# Autodesk Inventor assembly: HCMUTE-CDT23-PLXR_KXL
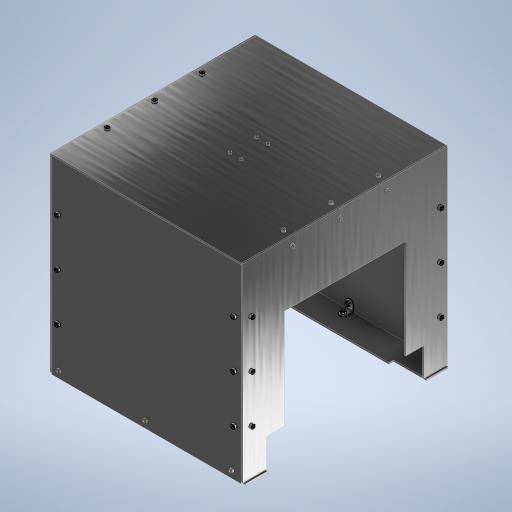
[picture p0: Inventor's stored thumbnail of the model, 512x512]
Saved by Autodesk Inventor 2023 (Build 270158000, 158)
## iProperties
Created: 2023-11-19
Part Number: HCMUTE-CDT23-PLXR_KXL
Document SubType Name: Assembly
Designer: havie
Mass: 52555 g
Surface Area: 83477.5 cm^2
Volume: 13075.1 cm^3
Density: 4.01946 g/cm^3
Author: havie
## Documents named in this file (15)
- D:\DO_AN_CDT\1.1. PART\HCMUTE-CDT23-PLXR_KXL.iam
- C:\Users\havie\Documents\Inventor\Content Center Files\R2023\en-US\ISO 4762(2)\ISO 4762 - M6 x 10ISO.ipt
- C:\Users\havie\Documents\Inventor\Content Center Files\R2023\en-US\ISO 4762(2)\ISO 4762 - M5 x 12ISO.ipt
- D:\DO_AN_CDT\1.1. PART\CAMERA\Assembly_HCMUTE-CDT23-CAMERA_C270Logitech c270 Assembly.iam
- D:\DO_AN_CDT\1.1. PART\HCMUTE-CDT23-KXL_A01.ipt
- C:\Users\havie\Documents\Inventor\Content Center Files\R2023\en-US\ISO 4032(2)\ISO 4032 - M5 - ISO.ipt
- D:\DO_AN_CDT\1.1. PART\2309HCMUTE-CDT23-KXL_GA-VUONG.ipt
- D:\DO_AN_CDT\1.1. PART\HCMUTE-CDT23-KXL_A02.ipt
- D:\DO_AN_CDT\1.1. PART\HCMUTE-CDT23-KXL_A03.ipt
- D:\DO_AN_CDT\1.1. PART\HCMUTE-CDT23-KXL_A04.ipt
- D:\DO_AN_CDT\1.1. PART\HCMUTE-CDT23-KXL_A05.ipt
- D:\DO_AN_CDT\1.1. PART\CBIEN\Assembly_HCMUTE-CDT23-CB_E3F-DS30C4.iam
- D:\DO_AN_CDT\1.1. PART\HCMUTE-CDT23-KXL_A06.ipt
- C:\Users\havie\Documents\Inventor\Content Center Files\R2023\en-US\ISO 4762(2)\ISO 4762 - M4 x 16ISO.ipt
- C:\Users\havie\Documents\Inventor\Content Center Files\R2023\en-US\ISO 4032(2)\ISO 4032 - M4 - ISO.ipt
## Components (144 placed, 14 different names)
1. HCMUTE-CDT23-KXL_A01:1 — Mate:288, Flush:55, Mate:289, Mate:290, Mate:291, Mate:292, Mate:293, Flush:57, Mate:313, Mate:360
2. 2309HCMUTE-CDT23-KXL_GA-VUONG:1 — Mate:288, Flush:55, Mate:289, Flush:56, Mate:476, Mate:477
3. 2309HCMUTE-CDT23-KXL_GA-VUONG:2 — Mate:290, Flush:56, Mate:291
4. 2309HCMUTE-CDT23-KXL_GA-VUONG:3 — Mate:292, Mate:293, Flush:57, Mate:478
5. ISO 4032 M5:1
6. HCMUTE-CDT23-KXL_A03:1 — Mate:313, Mate:316, Mate:319, Flush:61, Flush:62, Mate:338, Mate:355, Mate:356, Mate:370, Symmetry:3
7. HCMUTE-CDT23-KXL_A02:2 — Mate:319, Flush:61, Flush:62, Mate:333, Mate:334, Mate:335, Flush:69, Mate:336, Mate:337, Mate:341, Mate:342, Mate:347, Mate:348, Mate:351, Mate:352, Mate:474, Mate:475
8. HCMUTE-CDT23-KXL_A01:2 — Mate:331
9. HCMUTE-CDT23-KXL_A04:1 — Mate:360, Mate:361, Mate:362, Mate:363, Mate:364, Mate:373, Mate:380, Mate:381, Symmetry:3
10. HCMUTE-CDT23-KXL_A05:1 — Mate:370, Mate:371, Flush:72, Mate:372, Mate:374, Mate:375, Mate:382, Mate:383, Mate:384, Mate:385, Mate:386, Mate:481, Mate:482, Mate:483, Mate:484, Mate:485, Mate:486, Mate:487, Mate:488
11. ISO 4762 M5 x 12:44
12. ISO 4032 M5:40
13. ISO 4032 M5:41
14. ISO 4762 M5 x 12:45
15. ISO 4762 M5 x 12:46
16. ISO 4032 M5:42
17. ISO 4032 M5:43
18. ISO 4762 M5 x 12:47
19. ISO 4762 M5 x 12:48
20. ISO 4032 M5:44
21. ISO 4032 M5:45
22. ISO 4762 M5 x 12:49
23. Assembly_HCMUTE-CDT23-CAMERA_C270Logitech c270 Assembly:2 [sub-assembly] — Mate:384, Mate:385, Mate:386, Mate:493, Mate:494, Mate:495, Mate:496
24. Assembly_HCMUTE-CDT23-CB_E3F-DS30C4:2 [sub-assembly] — Mate:474, Mate:475
25. HCMUTE-CDT23-KXL_A06:1 — Mate:476, Mate:477, Mate:478
26. ISO 4032 M5:60 — Mate:479
27. ISO 4032 M5:61 — Mate:480
28. ISO 4762 M5 x 12:76 — Mate:480
29. ISO 4762 M5 x 12:77 — Mate:479
30. ISO 4032 M5:62
31. ISO 4032 M5:63
32. ISO 4762 M5 x 12:78
33. ISO 4762 M5 x 12:79
34. ISO 4032 M5:64
35. ISO 4032 M5:65
36. ISO 4762 M5 x 12:80
37. ISO 4762 M5 x 12:81
38. ISO 4762 M4 x 16:1 — Mate:483, Mate:486, Mate:490
39. ISO 4762 M4 x 16:2 — Mate:482, Mate:487, Mate:489
40. ISO 4762 M4 x 16:3 — Mate:481, Mate:488, Mate:491
41. ISO 4762 M4 x 16:4 — Mate:484, Mate:485, Mate:492
42. ISO 4032 M4:1 — Mate:489, Mate:494
43. ISO 4032 M4:2 — Mate:490, Mate:496
44. ISO 4032 M4:3 — Mate:491, Mate:493
45. ISO 4032 M4:4 — Mate:492, Mate:495
46. ISO 4032 M5:10 — Mate:317, Mate:318
47. ISO 4762 M5 x 12:14 — Mate:315, Mate:316, Mate:318
48. ISO 4032 M5:11
49. ISO 4762 M5 x 12:15
50. ISO 4032 M5:12
51. ISO 4762 M5 x 12:16
52. ISO 4762 M6 x 10:16
53. ISO 4762 M6 x 10:15
54. ISO 4762 M6 x 10:17
55. ISO 4762 M6 x 10:18
56. ISO 4762 M6 x 10:19
57. ISO 4762 M6 x 10:20
58. 2309HCMUTE-CDT23-KXL_GA-VUONG:10 — Mate:331, Mate:333, Mate:339, Mate:343, Mate:345
59. 2309HCMUTE-CDT23-KXL_GA-VUONG:13
60. 2309HCMUTE-CDT23-KXL_GA-VUONG:14
61. 2309HCMUTE-CDT23-KXL_GA-VUONG:11 — Mate:334, Mate:335, Flush:69, Mate:349
62. 2309HCMUTE-CDT23-KXL_GA-VUONG:12 — Mate:336, Mate:337, Mate:338, Mate:354, Mate:357
63. 2309HCMUTE-CDT23-KXL_GA-VUONG:15
64. 2309HCMUTE-CDT23-KXL_GA-VUONG:16
65. 2309HCMUTE-CDT23-KXL_GA-VUONG:17 — Mate:367
66. 2309HCMUTE-CDT23-KXL_GA-VUONG:18
67. ISO 4032 M5:15 — Mate:343, Mate:344
68. ISO 4032 M5:16 — Mate:345, Mate:346
69. ISO 4762 M5 x 12:20 — Mate:341, Mate:342, Mate:346
70. ISO 4762 M5 x 12:17 — Mate:339, Mate:344
71. ISO 4032 M5:17
72. ISO 4032 M5:18
73. ISO 4762 M5 x 12:21
74. ISO 4762 M5 x 12:22
75. ISO 4032 M5:19
76. ISO 4032 M5:20
77. ISO 4762 M5 x 12:23
78. ISO 4762 M5 x 12:24
79. ISO 4762 M5 x 12:18 — Mate:347, Mate:348, Mate:350
80. ISO 4032 M5:14 — Mate:349, Mate:350
81. ISO 4762 M5 x 12:25
82. ISO 4032 M5:21
83. ISO 4762 M5 x 12:26
84. ISO 4032 M5:22
85. ISO 4032 M5:13 — Mate:353, Mate:354
86. ISO 4762 M5 x 12:19 — Mate:351, Mate:352, Mate:353
87. ISO 4762 M5 x 12:27 — Mate:355, Mate:356, Mate:358
88. ISO 4032 M5:23 — Mate:357, Mate:358
89. ISO 4032 M5:24
90. ISO 4762 M5 x 12:28
91. ISO 4762 M5 x 12:29
92. ISO 4032 M5:25
93. ISO 4032 M5:26
94. ISO 4762 M5 x 12:30
95. ISO 4762 M5 x 12:31
96. ISO 4032 M5:27
97. ISO 4032 M5:29 — Mate:367, Mate:368
98. ISO 4762 M5 x 12:32 — Mate:361, Mate:362, Mate:368
99. ISO 4032 M5:28 — Mate:365, Mate:366
100. ISO 4762 M5 x 12:33 — Mate:363, Mate:364, Mate:366
101. ISO 4032 M5:30
102. ISO 4762 M5 x 12:34
103. ISO 4032 M5:31
104. ISO 4762 M5 x 12:35
105. ISO 4032 M5:32
106. ISO 4762 M5 x 12:36
107. ISO 4032 M5:33
108. ISO 4762 M5 x 12:37
109. 2309HCMUTE-CDT23-KXL_GA-VUONG:19 — Mate:371, Flush:72, Mate:372
110. 2309HCMUTE-CDT23-KXL_GA-VUONG:20
111. 2309HCMUTE-CDT23-KXL_GA-VUONG:21
112. 2309HCMUTE-CDT23-KXL_GA-VUONG:22 — Mate:373, Mate:374, Mate:375, Mate:376, Mate:377, Mate:378, Mate:379
113. 2309HCMUTE-CDT23-KXL_GA-VUONG:23
114. 2309HCMUTE-CDT23-KXL_GA-VUONG:24
115. ISO 4762 M5 x 12:38 — Mate:380, Mate:381
116. ISO 4032 M5:34 — Mate:376, Mate:377
117. ISO 4032 M5:35 — Mate:378, Mate:379
118. ISO 4762 M5 x 12:39 — Mate:382, Mate:383
119. ISO 4762 M5 x 12:40
120. ISO 4032 M5:36
121. ISO 4032 M5:37
122. ISO 4762 M5 x 12:41
123. ISO 4762 M5 x 12:42
124. ISO 4032 M5:38
125. ISO 4032 M5:39
126. ISO 4762 M5 x 12:43
127. 2309HCMUTE-CDT23-KXL_GA-VUONG:4 — Mate:309, Mate:365
128. ISO 4032 M5:5 — Mate:309, Mate:310
129. ISO 4762 M5 x 12:8 — Mate:310
130. 2309HCMUTE-CDT23-KXL_GA-VUONG:30
131. ISO 4032 M5:56
132. ISO 4762 M5 x 12:72
133. 2309HCMUTE-CDT23-KXL_GA-VUONG:31
134. ISO 4032 M5:57
135. ISO 4762 M5 x 12:73
136. ISO 4032 M5:4 — Mate:311, Mate:312
137. 2309HCMUTE-CDT23-KXL_GA-VUONG:7 — Mate:312, Mate:315, Mate:317
138. ISO 4762 M5 x 12:9 — Mate:311
139. ISO 4032 M5:58
140. 2309HCMUTE-CDT23-KXL_GA-VUONG:32
141. ISO 4762 M5 x 12:74
142. ISO 4032 M5:59
143. 2309HCMUTE-CDT23-KXL_GA-VUONG:33
144. ISO 4762 M5 x 12:75
## Component patterns: (3 elements, first: ISO 4032 M5:10 + ISO 4762 M5 x 12:14), (3 elements, first: ISO 4762 M6 x 10:16 + ISO 4762 M6 x 10:15), (3 elements, first: 2309HCMUTE-CDT23-KXL_GA-VUONG:10), (3 elements, first: 2309HCMUTE-CDT23-KXL_GA-VUONG:11 + 2309HCMUTE-CDT23-KXL_GA-VUONG:12), (3 elements, first: ISO 4032 M5:15 + ISO 4032 M5:16 + ISO 4762 M5 x 12:20 + ISO 4762 M5 x 12:17), (3 elements, first: ISO 4762 M5 x 12:18 + ISO 4032 M5:14), (3 elements, first: ISO 4032 M5:13 + ISO 4762 M5 x 12:19 + ISO 4762 M5 x 12:27 + ISO 4032 M5:23), (3 elements, first: ISO 4032 M5:29 + ISO 4762 M5 x 12:32 + ISO 4032 M5:28 + ISO 4762 M5 x 12:33), (3 elements, first: 2309HCMUTE-CDT23-KXL_GA-VUONG:19), (3 elements, first: 2309HCMUTE-CDT23-KXL_GA-VUONG:22), (3 elements, first: ISO 4762 M5 x 12:38 + ISO 4032 M5:34 + ISO 4032 M5:35 + ISO 4762 M5 x 12:39), (3 elements, first: 2309HCMUTE-CDT23-KXL_GA-VUONG:4 + ISO 4032 M5:5 + ISO 4762 M5 x 12:8), (3 elements, first: ISO 4032 M5:4 + 2309HCMUTE-CDT23-KXL_GA-VUONG:7 + ISO 4762 M5 x 12:9)
## Relationships (99: Mate 91, Flush 7, Symmetry 1)
- Mate:288: HCMUTE-CDT23-KXL_A01:1 ↔ 2309HCMUTE-CDT23-KXL_GA-VUONG:1
- Flush:55: HCMUTE-CDT23-KXL_A01:1 ↔ 2309HCMUTE-CDT23-KXL_GA-VUONG:1
- Mate:289: HCMUTE-CDT23-KXL_A01:1 ↔ 2309HCMUTE-CDT23-KXL_GA-VUONG:1
- Mate:290: HCMUTE-CDT23-KXL_A01:1 ↔ 2309HCMUTE-CDT23-KXL_GA-VUONG:2
- Flush:56: 2309HCMUTE-CDT23-KXL_GA-VUONG:1 ↔ 2309HCMUTE-CDT23-KXL_GA-VUONG:2
- Mate:291: HCMUTE-CDT23-KXL_A01:1 ↔ 2309HCMUTE-CDT23-KXL_GA-VUONG:2
- Mate:292: HCMUTE-CDT23-KXL_A01:1 ↔ 2309HCMUTE-CDT23-KXL_GA-VUONG:3
- Mate:293: HCMUTE-CDT23-KXL_A01:1 ↔ 2309HCMUTE-CDT23-KXL_GA-VUONG:3
- Flush:57: HCMUTE-CDT23-KXL_A01:1 ↔ 2309HCMUTE-CDT23-KXL_GA-VUONG:3
- Mate:309: 2309HCMUTE-CDT23-KXL_GA-VUONG:4 ↔ ISO 4032 M5:5
- Mate:310: ISO 4032 M5:5 ↔ ISO 4762 M5 x 12:8
- Mate:311: ISO 4032 M5:4 ↔ ISO 4762 M5 x 12:9
- Mate:312: ISO 4032 M5:4 ↔ 2309HCMUTE-CDT23-KXL_GA-VUONG:7
- Mate:313: HCMUTE-CDT23-KXL_A01:1 ↔ HCMUTE-CDT23-KXL_A03:1
- Mate:315: ISO 4762 M5 x 12:14 ↔ 2309HCMUTE-CDT23-KXL_GA-VUONG:7
- Mate:316: HCMUTE-CDT23-KXL_A03:1 ↔ ISO 4762 M5 x 12:14
- Mate:317: ISO 4032 M5:10 ↔ 2309HCMUTE-CDT23-KXL_GA-VUONG:7
- Mate:318: ISO 4032 M5:10 ↔ ISO 4762 M5 x 12:14
- Mate:319: HCMUTE-CDT23-KXL_A03:1 ↔ HCMUTE-CDT23-KXL_A02:2
- Flush:61: HCMUTE-CDT23-KXL_A03:1 ↔ HCMUTE-CDT23-KXL_A02:2
- Flush:62 (3 mm): HCMUTE-CDT23-KXL_A03:1 ↔ HCMUTE-CDT23-KXL_A02:2
- Mate:331: HCMUTE-CDT23-KXL_A01:2 ↔ 2309HCMUTE-CDT23-KXL_GA-VUONG:10
- Mate:333: HCMUTE-CDT23-KXL_A02:2 ↔ 2309HCMUTE-CDT23-KXL_GA-VUONG:10
- Mate:334: HCMUTE-CDT23-KXL_A02:2 ↔ 2309HCMUTE-CDT23-KXL_GA-VUONG:11
- Mate:335: HCMUTE-CDT23-KXL_A02:2 ↔ 2309HCMUTE-CDT23-KXL_GA-VUONG:11
- Flush:69: HCMUTE-CDT23-KXL_A02:2 ↔ 2309HCMUTE-CDT23-KXL_GA-VUONG:11
- Mate:336: HCMUTE-CDT23-KXL_A02:2 ↔ 2309HCMUTE-CDT23-KXL_GA-VUONG:12
- Mate:337: HCMUTE-CDT23-KXL_A02:2 ↔ 2309HCMUTE-CDT23-KXL_GA-VUONG:12
- Mate:338: HCMUTE-CDT23-KXL_A03:1 ↔ 2309HCMUTE-CDT23-KXL_GA-VUONG:12
- Mate:339: 2309HCMUTE-CDT23-KXL_GA-VUONG:10 ↔ ISO 4762 M5 x 12:17
- Mate:341: HCMUTE-CDT23-KXL_A02:2 ↔ ISO 4762 M5 x 12:20
- Mate:342: HCMUTE-CDT23-KXL_A02:2 ↔ ISO 4762 M5 x 12:20
- Mate:343: 2309HCMUTE-CDT23-KXL_GA-VUONG:10 ↔ ISO 4032 M5:15
- Mate:344: ISO 4032 M5:15 ↔ ISO 4762 M5 x 12:17
- Mate:345: 2309HCMUTE-CDT23-KXL_GA-VUONG:10 ↔ ISO 4032 M5:16
- Mate:346: ISO 4032 M5:16 ↔ ISO 4762 M5 x 12:20
- Mate:347: HCMUTE-CDT23-KXL_A02:2 ↔ ISO 4762 M5 x 12:18
- Mate:348: HCMUTE-CDT23-KXL_A02:2 ↔ ISO 4762 M5 x 12:18
- Mate:349: 2309HCMUTE-CDT23-KXL_GA-VUONG:11 ↔ ISO 4032 M5:14
- Mate:350: ISO 4762 M5 x 12:18 ↔ ISO 4032 M5:14
- Mate:351: HCMUTE-CDT23-KXL_A02:2 ↔ ISO 4762 M5 x 12:19
- Mate:352: HCMUTE-CDT23-KXL_A02:2 ↔ ISO 4762 M5 x 12:19
- Mate:353: ISO 4032 M5:13 ↔ ISO 4762 M5 x 12:19
- Mate:354: 2309HCMUTE-CDT23-KXL_GA-VUONG:12 ↔ ISO 4032 M5:13
- Mate:355: HCMUTE-CDT23-KXL_A03:1 ↔ ISO 4762 M5 x 12:27
- Mate:356: HCMUTE-CDT23-KXL_A03:1 ↔ ISO 4762 M5 x 12:27
- Mate:357: 2309HCMUTE-CDT23-KXL_GA-VUONG:12 ↔ ISO 4032 M5:23
- Mate:358: ISO 4762 M5 x 12:27 ↔ ISO 4032 M5:23
- Mate:360: HCMUTE-CDT23-KXL_A01:1 ↔ HCMUTE-CDT23-KXL_A04:1
- Mate:361: HCMUTE-CDT23-KXL_A04:1 ↔ ISO 4762 M5 x 12:32
- Mate:362: HCMUTE-CDT23-KXL_A04:1 ↔ ISO 4762 M5 x 12:32
- Mate:363: HCMUTE-CDT23-KXL_A04:1 ↔ ISO 4762 M5 x 12:33
- Mate:364: HCMUTE-CDT23-KXL_A04:1 ↔ ISO 4762 M5 x 12:33
- Mate:365: ISO 4032 M5:28 ↔ 2309HCMUTE-CDT23-KXL_GA-VUONG:4
- Mate:366: ISO 4032 M5:28 ↔ ISO 4762 M5 x 12:33
- Mate:367: 2309HCMUTE-CDT23-KXL_GA-VUONG:17 ↔ ISO 4032 M5:29
- Mate:368: ISO 4032 M5:29 ↔ ISO 4762 M5 x 12:32
- Mate:370: HCMUTE-CDT23-KXL_A03:1 ↔ HCMUTE-CDT23-KXL_A05:1
- Mate:371: HCMUTE-CDT23-KXL_A05:1 ↔ 2309HCMUTE-CDT23-KXL_GA-VUONG:19
- Flush:72: HCMUTE-CDT23-KXL_A05:1 ↔ 2309HCMUTE-CDT23-KXL_GA-VUONG:19
- Mate:372: HCMUTE-CDT23-KXL_A05:1 ↔ 2309HCMUTE-CDT23-KXL_GA-VUONG:19
- Mate:373: HCMUTE-CDT23-KXL_A04:1 ↔ 2309HCMUTE-CDT23-KXL_GA-VUONG:22
- Mate:374: HCMUTE-CDT23-KXL_A05:1 ↔ 2309HCMUTE-CDT23-KXL_GA-VUONG:22
- Mate:375: HCMUTE-CDT23-KXL_A05:1 ↔ 2309HCMUTE-CDT23-KXL_GA-VUONG:22
- Mate:376: 2309HCMUTE-CDT23-KXL_GA-VUONG:22 ↔ ISO 4032 M5:34
- Mate:377: 2309HCMUTE-CDT23-KXL_GA-VUONG:22 ↔ ISO 4032 M5:34
- Mate:378: 2309HCMUTE-CDT23-KXL_GA-VUONG:22 ↔ ISO 4032 M5:35
- Mate:379: 2309HCMUTE-CDT23-KXL_GA-VUONG:22 ↔ ISO 4032 M5:35
- Mate:380: HCMUTE-CDT23-KXL_A04:1 ↔ ISO 4762 M5 x 12:38
- Mate:381: HCMUTE-CDT23-KXL_A04:1 ↔ ISO 4762 M5 x 12:38
- Mate:382: HCMUTE-CDT23-KXL_A05:1 ↔ ISO 4762 M5 x 12:39
- Mate:383: HCMUTE-CDT23-KXL_A05:1 ↔ ISO 4762 M5 x 12:39
- Symmetry:3: HCMUTE-CDT23-KXL_A03:1 ↔ HCMUTE-CDT23-KXL_A04:1
- Mate:384: HCMUTE-CDT23-KXL_A05:1 ↔ Assembly_HCMUTE-CDT23-CAMERA_C270Logitech c270 Assembly:2
- Mate:385: HCMUTE-CDT23-KXL_A05:1 ↔ Assembly_HCMUTE-CDT23-CAMERA_C270Logitech c270 Assembly:2
- Mate:386: HCMUTE-CDT23-KXL_A05:1 ↔ Assembly_HCMUTE-CDT23-CAMERA_C270Logitech c270 Assembly:2
- Mate:474: HCMUTE-CDT23-KXL_A02:2 ↔ Assembly_HCMUTE-CDT23-CB_E3F-DS30C4:2
- Mate:475: HCMUTE-CDT23-KXL_A02:2 ↔ Assembly_HCMUTE-CDT23-CB_E3F-DS30C4:2
- Mate:476: 2309HCMUTE-CDT23-KXL_GA-VUONG:1 ↔ HCMUTE-CDT23-KXL_A06:1
- Mate:477: 2309HCMUTE-CDT23-KXL_GA-VUONG:1 ↔ HCMUTE-CDT23-KXL_A06:1
- Mate:478: 2309HCMUTE-CDT23-KXL_GA-VUONG:3 ↔ HCMUTE-CDT23-KXL_A06:1
- Mate:479: ISO 4032 M5:60 ↔ ISO 4762 M5 x 12:77
- Mate:480: ISO 4032 M5:61 ↔ ISO 4762 M5 x 12:76
- Mate:481: HCMUTE-CDT23-KXL_A05:1 ↔ ISO 4762 M4 x 16:3
- Mate:482: HCMUTE-CDT23-KXL_A05:1 ↔ ISO 4762 M4 x 16:2
- Mate:483: HCMUTE-CDT23-KXL_A05:1 ↔ ISO 4762 M4 x 16:1
- Mate:484: HCMUTE-CDT23-KXL_A05:1 ↔ ISO 4762 M4 x 16:4
- Mate:485: HCMUTE-CDT23-KXL_A05:1 ↔ ISO 4762 M4 x 16:4
- Mate:486: HCMUTE-CDT23-KXL_A05:1 ↔ ISO 4762 M4 x 16:1
- Mate:487: HCMUTE-CDT23-KXL_A05:1 ↔ ISO 4762 M4 x 16:2
- Mate:488: HCMUTE-CDT23-KXL_A05:1 ↔ ISO 4762 M4 x 16:3
- Mate:489: ISO 4762 M4 x 16:2 ↔ ISO 4032 M4:1
- Mate:490: ISO 4762 M4 x 16:1 ↔ ISO 4032 M4:2
- Mate:491: ISO 4762 M4 x 16:3 ↔ ISO 4032 M4:3
- Mate:492: ISO 4762 M4 x 16:4 ↔ ISO 4032 M4:4
- Mate:493: Assembly_HCMUTE-CDT23-CAMERA_C270Logitech c270 Assembly:2 ↔ ISO 4032 M4:3
- Mate:494: Assembly_HCMUTE-CDT23-CAMERA_C270Logitech c270 Assembly:2 ↔ ISO 4032 M4:1
- Mate:495: Assembly_HCMUTE-CDT23-CAMERA_C270Logitech c270 Assembly:2 ↔ ISO 4032 M4:4
- Mate:496: Assembly_HCMUTE-CDT23-CAMERA_C270Logitech c270 Assembly:2 ↔ ISO 4032 M4:2
